# Autodesk Inventor assembly: board_setter
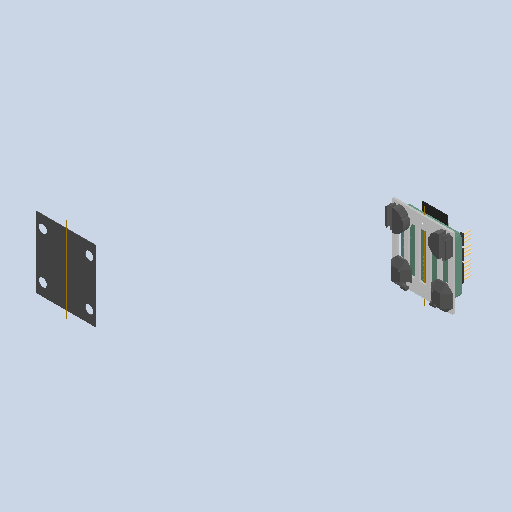
[picture p0: Inventor's stored thumbnail of the model, 512x512]
Saved by Autodesk Inventor 2026.1 (Build 301233020, 233B)
## iProperties
Created: 2024-10-09
Part Number: board_setter
Document SubType Name: Assembly
Designer: hibik
Author: hibik
## Documents named in this file (6)
- C:\Users\hibik\Documents\Robomech\HR\Eglantyne_mark2\hard\under_body\board_setter\board_setter.iam
- C:\Users\hibik\Documents\Robomech\HR\Eglantyne_mark2\hard\under_body\board_setter\board_setter_base.ipt
- C:\Users\hibik\Documents\Robomech\HR\Eglantyne_mark2\hard\needed_model\ControlBoard.iam
- C:\Users\hibik\Documents\Robomech\HR\Eglantyne_mark2\hard\under_body\board_setter\board_setter_cover_under.ipt
- C:\Users\hibik\Documents\Robomech\HR\Eglantyne_mark2\hard\under_body\board_setter\board_setter_upper.ipt
- C:\Users\hibik\Documents\Robomech\HR\Eglantyne_mark2\hard\under_body\board_setter\board_setter_safety.ipt
## Components (5 placed, 5 different names)
1. board_setter_base:1 — 挿入:1, 挿入:2, 角度:1, メイト:1
2. ControlBoard:1 [sub-assembly] — 挿入:3, 角度:1
3. board_setter_cover_under:1 — 挿入:1, 挿入:2, 挿入:3
4. board_setter_upper:1 — メイト:1
5. board_setter_safety:1
## Relationships (5: Insert 3, Angle 1, Mate 1)
- 挿入:1 [Insert]: board_setter_base:1 ↔ board_setter_cover_under:1
- 挿入:2 [Insert]: board_setter_base:1 ↔ board_setter_cover_under:1
- 挿入:3 [Insert]: ControlBoard:1 ↔ board_setter_cover_under:1
- 角度:1 [Angle] (0 deg): board_setter_base:1 ↔ ControlBoard:1
- メイト:1 [Mate]: board_setter_base:1 ↔ board_setter_upper:1
